# Autodesk Inventor assembly: Whole-body-cuvette-30x30x120
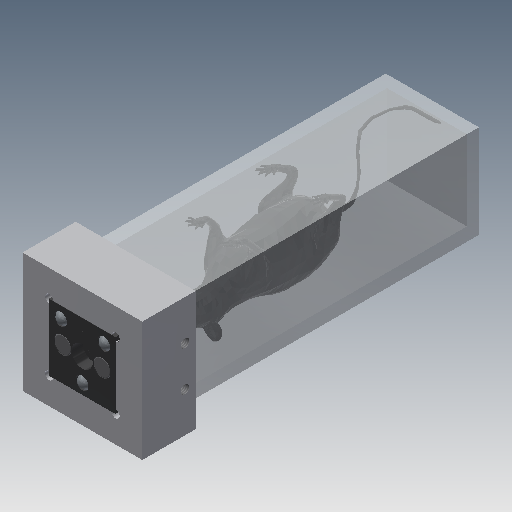
[picture p0: Inventor's stored thumbnail of the model, 512x512]
Saved by Autodesk Inventor 2021 (Build 250183000, 183)
## iProperties
Created: 2019-09-25
Part Number: Whole-body-cuvette-30x30x120
Document SubType Name: Assembly
Designer: voigt
Author: voigt
## Documents named in this file (5)
- C:\Users\Public\GitHub-public\benchtop-hardware\Benchtop\CAD-model-Inventor2021\mesoSPIM\sample_handling\assemblies\whole-mouse-cuvette-30x30x120.iam
- C:\Users\Public\GitHub-public\benchtop-hardware\Benchtop\CAD-model-Inventor2021\library\Portmann Instruments\UG-752-30x30x120mm.ipt
- C:\Users\Public\GitHub-public\benchtop-hardware\Benchtop\CAD-model-Inventor2021\mesoSPIM\immersion_cuvette_mounts\Large-cuvette-mount-30mm-V1.ipt
- C:\Users\Public\GitHub-public\benchtop-hardware\Benchtop\CAD-model-Inventor2021\library\Thorlabs\kinematic_bases\KBT25_top_steelballs_simplified.ipt
- C:\Users\Public\GitHub-public\benchtop-hardware\Benchtop\CAD-model-Inventor2021\library\samples\mouse10cm-curled-tail.ipt
## Components (4 placed, 4 different names)
1. UG-752-30x30x120mm:1 — Mate:1, Flush:1, Mate:2, Mate:3, Mate:4, Mate:5
2. Large-cuvette-mount-30mm-V1:1 — Mate:3, Mate:4, Mate:5, Mate:6, Mate:7, Mate:8
3. KBT25_top_steelballs_simplified:1 — Mate:6, Mate:7, Mate:8
4. mouse10cm-curled-tail:1
## Relationships (9: Mate 8, Flush 1)
- Mate:1: UG-752-30x30x120mm:1
- Flush:1 (-17.5 mm): UG-752-30x30x120mm:1
- Mate:2 (-17.5 mm): UG-752-30x30x120mm:1
- Mate:3: UG-752-30x30x120mm:1 ↔ Large-cuvette-mount-30mm-V1:1
- Mate:4: UG-752-30x30x120mm:1 ↔ Large-cuvette-mount-30mm-V1:1
- Mate:5: UG-752-30x30x120mm:1 ↔ Large-cuvette-mount-30mm-V1:1
- Mate:6: Large-cuvette-mount-30mm-V1:1 ↔ KBT25_top_steelballs_simplified:1
- Mate:7: Large-cuvette-mount-30mm-V1:1 ↔ KBT25_top_steelballs_simplified:1
- Mate:8: Large-cuvette-mount-30mm-V1:1 ↔ KBT25_top_steelballs_simplified:1
